(part 1 of 2)
# Autodesk Inventor assembly: robot
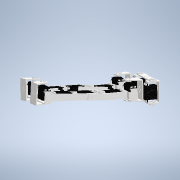
[picture p0: Inventor's stored thumbnail of the model, 180x180]
Saved by Autodesk Inventor 2021.4 (Build 254397000, 397)
## iProperties
Created: 2022-07-17
Part Number: robot
Document SubType Name: Assembly
Designer: isamu
Author: isamu
## Documents named in this file (28)
- D:\personal_projects\robot\inventor\2021-exportable\robot.iam
- D:\personal_projects\robot\exports\servo motors\servo-motor-mg996r servo.ipt
- D:\personal_projects\robot\exports\frames\servo frame.ipt
- D:\personal_projects\robot\exports\handle\servo handle 4.ipt
- D:\personal_projects\robot\exports\screws\m4x8.ipt
- D:\personal_projects\robot\exports\screws\m4 nuts.ipt
- D:\personal_projects\robot\exports\screws\m4x12.ipt
- D:\personal_projects\robot\exports\frames\servo frame mg996r.ipt
- D:\personal_projects\robot\exports\screws\m2x8.ipt
- D:\personal_projects\robot\exports\screws\m2 nuts.ipt
- D:\personal_projects\robot\exports\frames\servo frame part 3.ipt
- D:\personal_projects\robot\exports\frames\servo frame mg996 centered_MIR.ipt
- D:\personal_projects\robot\exports\frames\servo frame mg996 foot_MIR.ipt
- D:\personal_projects\robot\exports\frames\servo frame part 4.ipt
- D:\personal_projects\robot\exports\servo motors\servo-motor-mg996r servo_MIR.ipt
- D:\personal_projects\robot\exports\frames\servo frame_MIR.ipt
- D:\personal_projects\robot\exports\screws\m4x8_MIR.ipt
- D:\personal_projects\robot\exports\screws\m4 nuts_MIR.ipt
- D:\personal_projects\robot\exports\screws\m4x12_MIR.ipt
- D:\personal_projects\robot\exports\frames\servo frame mg996r_MIR.ipt
- D:\personal_projects\robot\exports\handle\servo handle 4_MIR.ipt
- D:\personal_projects\robot\exports\screws\m2x8_MIR.ipt
- D:\personal_projects\robot\exports\screws\m2 nuts_MIR.ipt
- D:\personal_projects\robot\exports\frames\servo frame part 3_MIR.ipt
- D:\personal_projects\robot\exports\frames\servo frame mg996 centered_MIR_MIR.ipt
- D:\personal_projects\robot\exports\frames\servo frame mg996 foot_MIR_MIR.ipt
- D:\personal_projects\robot\exports\screws\m3x8.ipt
- D:\personal_projects\robot\exports\screws\m3 nuts.ipt
## Components (474 placed, 27 different names)
1. servo-motor-mg996r servo:1 — Mate:1, Mate:2, Mate:3, Insert:1, Insert:2, Insert:3, Insert:4, Rotational:1
2. servo frame:1 — Mate:1, Mate:2, Mate:3, Insert:5, Insert:6, Insert:7, Insert:8, Insert:9, Insert:10, Mate:32, Mate:33, Mate:34, Insert:376, Insert:377, Insert:378, Insert:379, Insert:380
3. m4x8:1 — Insert:2
4. m4x8:2 — Insert:3
5. m4x8:3 — Insert:4
6. m4x8:4 — Insert:1
7. m4 nuts:1 — Insert:5
8. m4 nuts:2 — Insert:6
9. m4 nuts:3 — Insert:7
10. m4 nuts:4 — Insert:8
11. m4x12:1 — Insert:9
12. m4 nuts:5 — Insert:10
13. servo frame mg996r:1 — Mate:4, Mate:5, Mate:6, Insert:11, Insert:16, Insert:17, Insert:18, Insert:19, Mate:13, Mate:14, Mate:15, Mate:16, Insert:281, Insert:282, Insert:283, Insert:284, Insert:285
14. servo handle 4:1 — Rotational:1, Mate:4, Mate:5, Mate:6, Insert:12, Insert:13, Insert:14, Insert:15
15. m4 nuts:6 — Insert:11
16. m2x8:1 — Insert:12
17. m2x8:2 — Insert:13
18. m2x8:3 — Insert:15
19. m2x8:4 — Insert:14
20. m2 nuts:1 — Insert:19
21. m2 nuts:2 — Insert:18
22. m2 nuts:3 — Insert:16
23. m2 nuts:4 — Insert:17
24. servo-motor-mg996r servo:2
25. servo frame:2 — Mate:23, Mate:24, Mate:25, Insert:291, Insert:292, Insert:293, Insert:294, Insert:295
26. m4x8:5
27. m4x8:6
28. m4x8:7
29. m4x8:8
30. m4 nuts:7
31. m4 nuts:8
32. m4 nuts:9
33. m4 nuts:10
34. m4x12:2
35. m4 nuts:11
36. servo frame mg996r:2 — Mate:13, Mate:14, Mate:15, Mate:16, Insert:386, Insert:387, Insert:388, Insert:389, Insert:390
37. servo handle 4:2
38. m4 nuts:12
39. m2x8:5
40. m2x8:6
41. m2x8:7
42. m2x8:8
43. m2 nuts:5
44. m2 nuts:6
45. m2 nuts:7
46. m2 nuts:8
47. servo-motor-mg996r servo:3
48. servo frame:3 — Mate:23, Mate:24, Mate:25, Insert:396, Insert:397, Insert:398, Insert:399, Insert:400
49. m4x8:9
50. m4x8:10
51. m4x8:11
52. m4x8:12
53. m4 nuts:13
54. m4 nuts:14
55. m4 nuts:15
56. m4 nuts:16
57. m4x12:3
58. m4 nuts:17
59. servo frame mg996r:3 — Mate:44, Mate:45, Mate:46, Mate:47, Insert:296, Insert:297, Insert:298, Insert:299, Insert:300
60. servo handle 4:3
61. m4 nuts:18
62. m2x8:9
63. m2x8:10
64. m2x8:11
65. m2x8:12
66. m2 nuts:9
67. m2 nuts:10
68. m2 nuts:11
69. m2 nuts:12
70. servo-motor-mg996r servo:4
71. servo frame:4 — Mate:29, Mate:30, Mate:31, Insert:406, Insert:407, Insert:408, Insert:409, Insert:410, Insert:411, Insert:412, Insert:413, Insert:414, Insert:415
72. m4x8:13
73. m4x8:14
74. m4x8:15
75. m4x8:16
76. m4 nuts:19
77. m4 nuts:20
78. m4 nuts:21
79. m4 nuts:22
80. m4x12:4 — Mate:36
81. m4 nuts:23
82. servo handle 4:4 — Mate:35
83. m2x8:13
84. m2x8:14
85. m2x8:15
86. m2x8:16 — Mate:37
87. servo frame part 3:1 — Mate:29, Mate:30, Mate:31, Mate:32, Mate:33, Mate:34, Insert:286, Insert:287, Insert:288, Insert:289, Insert:290, Insert:316, Insert:317, Insert:318, Insert:319, Insert:320, Insert:321, Insert:322, Insert:323, Insert:324, Insert:325
88. servo frame mg996 centered_MIR:1 — Mate:35, Mate:36, Mate:37, Mate:54, Mate:55, Mate:56, Mate:146, Insert:456, Insert:468, Insert:469, Insert:470, Insert:471, Insert:476, Insert:477, Insert:478, Insert:479
89. servo-motor-mg996r servo:5
90. servo frame:5 — Mate:41, Mate:42, Mate:43, Insert:436, Insert:437, Insert:438, Insert:439, Insert:440, Insert:446, Insert:447, Insert:448, Insert:449, Insert:450
91. m4x8:17
92. m4x8:18
93. m4x8:19
94. m4x8:20
95. m4 nuts:24
96. m4 nuts:25
97. m4 nuts:26
98. m4 nuts:27
99. m4x12:5
100. m4 nuts:28
101. servo handle 4:5 — Mate:50
102. m2x8:17
103. m2x8:18 — Mate:49
104. m2x8:19 — Mate:48
105. m2x8:20
106. servo frame part 3:2 — Mate:41, Mate:42, Mate:43, Mate:44, Mate:45, Mate:46, Mate:47, Insert:346, Insert:347, Insert:348, Insert:349, Insert:350, Insert:351, Insert:352, Insert:353, Insert:354, Insert:355, Insert:426, Insert:430, Insert:431, Insert:432, Insert:433
107. servo frame mg996 foot_MIR:1 — Mate:48, Mate:49, Mate:50, Insert:458, Insert:460, Insert:461, Insert:462, Insert:463
108. servo-motor-mg996r servo:6
109. servo frame:6 — Mate:57, Mate:58, Mate:59, Mate:60, Mate:61, Mate:62, Insert:356, Insert:357, Insert:358, Insert:359, Insert:360, Insert:361, Insert:362, Insert:363, Insert:364, Insert:365
110. m4x8:21
111. m4x8:22
112. m4x8:23
113. m4x8:24
114. m4 nuts:29
115. m4 nuts:30
116. m4 nuts:31
117. m4 nuts:32
118. servo handle 4:6 — Mate:54
119. m2x8:21 — Mate:56
120. m2x8:22
121. m2x8:23 — Mate:146
122. m2x8:24 — Mate:55
123. servo frame part 4:1 — Mate:57, Mate:58, Mate:59, Mate:91, Mate:92, Mate:93, Insert:256, Insert:257, Insert:258, Insert:259, Insert:260, Insert:271, Insert:272, Insert:273, Insert:274, Insert:275
124. servo frame part 4:2 — Mate:60, Mate:61, Mate:62, Insert:261, Insert:262, Insert:263, Insert:264, Insert:265, Insert:266, Insert:267, Insert:268, Insert:269, Insert:270
125. servo-motor-mg996r servo:10
126. servo frame:10 — Mate:91, Mate:92, Mate:93, Insert:366, Insert:367, Insert:368, Insert:369, Insert:370, Insert:371, Insert:372, Insert:373, Insert:374, Insert:375
127. m4x8:37
128. m4x8:38
129. m4x8:39
130. m4x8:40
131. m4 nuts:51
132. m4 nuts:52
133. m4 nuts:53
134. m4 nuts:54
135. servo handle 4:10 — Mate:144, Insert:252, Insert:253, Insert:254, Insert:255
136. servo-motor-mg996r servo_MIR:1 — Mate:94, Mate:95, Mate:96, Insert:167, Insert:168, Insert:169, Insert:170, Rotational:11
137. servo frame_MIR:1 — Mate:94, Mate:95, Mate:96, Insert:171, Insert:172, Insert:173, Insert:174, Insert:175, Insert:176, Mate:122, Mate:123, Mate:124, Insert:381, Insert:382, Insert:383, Insert:384, Insert:385
138. m4x8_MIR:1 — Insert:167
139. m4x8_MIR:2 — Insert:168
140. m4x8_MIR:3 — Insert:169
141. m4x8_MIR:4 — Insert:170
142. m4 nuts_MIR:1 — Insert:171
143. m4 nuts_MIR:2 — Insert:172
144. m4 nuts_MIR:3 — Insert:173
145. m4 nuts_MIR:4 — Insert:174
146. m4x12_MIR:1 — Insert:175
147. m4 nuts_MIR:5 — Insert:176
148. servo frame mg996r_MIR:1 — Mate:97, Mate:98, Mate:99, Insert:177, Insert:182, Insert:183, Insert:184, Insert:185, Mate:103, Mate:104, Mate:105, Mate:106, Insert:276, Insert:277, Insert:278, Insert:279, Insert:280
149. servo handle 4_MIR:1 — Mate:97, Mate:98, Mate:99, Insert:178, Insert:179, Insert:180, Insert:181, Rotational:11
150. m4 nuts_MIR:6 — Insert:177
151. m2x8_MIR:1 — Insert:178
152. m2x8_MIR:2 — Insert:179
153. m2x8_MIR:3 — Insert:180
154. m2x8_MIR:4 — Insert:181
155. m2 nuts_MIR:1 — Insert:182
156. m2 nuts_MIR:2 — Insert:183
157. m2 nuts_MIR:3 — Insert:184
158. m2 nuts_MIR:4 — Insert:185
159. servo-motor-mg996r servo_MIR:2 — Mate:100, Mate:101, Mate:102, Insert:186, Insert:187, Insert:188, Insert:189, Rotational:12
160. servo frame_MIR:2 — Mate:100, Mate:101, Mate:102, Insert:190, Insert:191, Insert:192, Insert:193, Insert:194, Insert:195, Mate:110, Mate:111, Mate:112, Insert:306, Insert:307, Insert:308, Insert:309, Insert:310
161. m4x8_MIR:5 — Insert:186
162. m4x8_MIR:6 — Insert:187
163. m4x8_MIR:7 — Insert:188
164. m4x8_MIR:8 — Insert:189
165. m4 nuts_MIR:7 — Insert:190
166. m4 nuts_MIR:8 — Insert:191
167. m4 nuts_MIR:9 — Insert:192
168. m4 nuts_MIR:10 — Insert:193
169. m4x12_MIR:2 — Insert:194
170. m4 nuts_MIR:11 — Insert:195
171. servo frame mg996r_MIR:2 — Mate:103, Mate:104, Mate:105, Mate:106, Mate:107, Mate:108, Mate:109, Insert:196, Insert:201, Insert:202, Insert:203, Insert:204, Insert:391, Insert:392, Insert:393, Insert:394, Insert:395
172. servo handle 4_MIR:2 — Mate:107, Mate:108, Mate:109, Insert:197, Insert:198, Insert:199, Insert:200, Rotational:12
173. m4 nuts_MIR:12 — Insert:196
174. m2x8_MIR:5 — Insert:197
175. m2x8_MIR:6 — Insert:198
176. m2x8_MIR:7 — Insert:199
177. m2x8_MIR:8 — Insert:200
178. m2 nuts_MIR:5 — Insert:201
179. m2 nuts_MIR:6 — Insert:202
180. m2 nuts_MIR:7 — Insert:203
181. m2 nuts_MIR:8 — Insert:204
182. servo-motor-mg996r servo_MIR:3 — Mate:113, Mate:114, Mate:115, Insert:205, Insert:206, Insert:207, Insert:208, Rotational:13
183. servo frame_MIR:3 — Mate:110, Mate:111, Mate:112, Mate:113, Mate:114, Mate:115, Insert:209, Insert:210, Insert:211, Insert:212, Insert:213, Insert:214, Insert:401, Insert:402, Insert:403, Insert:404, Insert:405
184. m4x8_MIR:9 — Insert:205
185. m4x8_MIR:10 — Insert:206
186. m4x8_MIR:11 — Insert:207
187. m4x8_MIR:12 — Insert:208
188. m4 nuts_MIR:13 — Insert:209
189. m4 nuts_MIR:14 — Insert:210
190. m4 nuts_MIR:15 — Insert:211
191. m4 nuts_MIR:16 — Insert:212
192. m4x12_MIR:3 — Insert:213
193. m4 nuts_MIR:17 — Insert:214
194. servo frame mg996r_MIR:3 — Mate:116, Mate:117, Mate:118, Insert:215, Insert:220, Insert:221, Insert:222, Insert:223, Mate:134, Mate:135, Mate:136, Mate:137, Insert:301, Insert:302, Insert:303, Insert:304, Insert:305
195. servo handle 4_MIR:3 — Mate:116, Mate:117, Mate:118, Insert:216, Insert:217, Insert:218, Insert:219, Rotational:13
196. m4 nuts_MIR:18 — Insert:215
197. m2x8_MIR:9 — Insert:216
198. m2x8_MIR:10 — Insert:217
199. m2x8_MIR:11 — Insert:218
200. m2x8_MIR:12 — Insert:219
201. m2 nuts_MIR:9 — Insert:220
202. m2 nuts_MIR:10 — Insert:221
203. m2 nuts_MIR:11 — Insert:222
204. m2 nuts_MIR:12 — Insert:223
205. servo-motor-mg996r servo_MIR:4 — Mate:119, Mate:120, Mate:121, Insert:224, Insert:225, Insert:226, Insert:227, Rotational:14
206. servo frame_MIR:4 — Mate:119, Mate:120, Mate:121, Insert:228, Insert:229, Insert:230, Insert:231, Insert:232, Insert:233, Mate:125, Mate:126, Mate:127, Insert:416, Insert:417, Insert:418, Insert:419, Insert:420, Insert:421, Insert:422, Insert:423, Insert:424, Insert:425
207. m4x8_MIR:13 — Insert:224
208. m4x8_MIR:14 — Insert:225
209. m4x8_MIR:15 — Insert:226
210. m4x8_MIR:16 — Insert:227
211. m4 nuts_MIR:19 — Insert:228
212. m4 nuts_MIR:20 — Insert:229
213. m4 nuts_MIR:21 — Insert:230
214. m4 nuts_MIR:22 — Insert:231
215. m4x12_MIR:4 — Insert:232, Mate:129
216. m4 nuts_MIR:23 — Insert:233
217. servo handle 4_MIR:4 — Insert:234, Insert:235, Insert:236, Insert:237, Mate:130, Rotational:14
218. m2x8_MIR:13 — Insert:234
219. m2x8_MIR:14 — Insert:235
220. m2x8_MIR:15 — Insert:236
221. m2x8_MIR:16 — Insert:237, Mate:128
222. servo frame part 3_MIR:1 — Mate:122, Mate:123, Mate:124, Mate:125, Mate:126, Mate:127, Insert:311, Insert:312, Insert:313, Insert:314, Insert:315, Insert:326, Insert:327, Insert:328, Insert:329, Insert:330, Insert:331, Insert:332, Insert:333, Insert:334, Insert:335
223. servo frame mg996 centered_MIR_MIR:1 — Mate:128, Mate:129, Mate:130, Mate:144, Mate:147, Mate:148, Insert:457, Insert:472, Insert:473, Insert:474, Insert:475, Insert:480, Insert:481, Insert:482, Insert:483
224. servo-motor-mg996r servo_MIR:5 — Mate:131, Mate:132, Mate:133, Insert:238, Insert:239, Insert:240, Insert:241, Rotational:15
225. servo frame_MIR:5 — Mate:131, Mate:132, Mate:133, Insert:242, Insert:243, Insert:244, Insert:245, Insert:246, Insert:247, Mate:138, Mate:139, Mate:140, Insert:441, Insert:442, Insert:443, Insert:444, Insert:445, Insert:451, Insert:452, Insert:453, Insert:454, Insert:455
226. m4x8_MIR:17 — Insert:238
227. m4x8_MIR:18 — Insert:239
228. m4x8_MIR:19 — Insert:240
229. m4x8_MIR:20 — Insert:241
230. m4 nuts_MIR:24 — Insert:242
231. m4 nuts_MIR:25 — Insert:243
232. m4 nuts_MIR:26 — Insert:244
233. m4 nuts_MIR:27 — Insert:245
234. m4x12_MIR:5 — Insert:246
235. m4 nuts_MIR:28 — Insert:247
236. servo handle 4_MIR:5 — Insert:248, Insert:249, Insert:250, Insert:251, Mate:141, Rotational:15
237. m2x8_MIR:17 — Insert:248
238. m2x8_MIR:18 — Insert:249, Mate:142
239. m2x8_MIR:19 — Insert:250, Mate:143
240. m2x8_MIR:20 — Insert:251
241. servo frame part 3_MIR:2 — Mate:134, Mate:135, Mate:136, Mate:137, Mate:138, Mate:139, Mate:140, Insert:336, Insert:337, Insert:338, Insert:339, Insert:340, Insert:341, Insert:342, Insert:343, Insert:344, Insert:345, Insert:427, Insert:428, Insert:429, Insert:434, Insert:435
242. servo frame mg996 foot_MIR_MIR:1 — Mate:141, Mate:142, Mate:143, Insert:459, Insert:464, Insert:465, Insert:466, Insert:467
243. m2x8:41 — Insert:252
244. m2x8:42 — Insert:255, Mate:148
245. m2x8:43 — Insert:253, Mate:147
246. m2x8:44 — Insert:254
247. m3x8:1 — Insert:269
248. m3x8:2 — Insert:270
249. m3x8:3 — Insert:265
250. m3x8:4 — Insert:264
251. m3x8:5 — Insert:266
252. m3x8:6 — Insert:276
253. m3x8:7 — Insert:277
254. m3x8:8 — Insert:278
255. m3x8:9 — Insert:274
256. m3x8:10 — Insert:275
257. m3x8:11 — Insert:271
258. m3x8:12 — Insert:284
259. m3x8:13 — Insert:283
260. m3x8:14 — Insert:282
261. m3x8:15 — Insert:281
262. m3x8:16 — Insert:259
263. m3x8:17 — Insert:260
264. m3x8:18 — Insert:258
265. m3x8:19 — Insert:257
266. m3x8:20 — Insert:256
267. m3x8:21 — Insert:280
268. m3x8:22 — Insert:285
269. m3x8:23 — Insert:279
270. m3x8:24 — Insert:272
271. m3x8:25 — Insert:273
272. m3x8:26 — Insert:290
273. m3x8:27 — Insert:289
274. m3x8:28 — Insert:288
275. m3x8:29 — Insert:287
276. m3x8:30 — Insert:286
277. m3x8:31 — Insert:306
278. m3x8:32 — Insert:330
279. m3x8:33 — Insert:329
280. m3x8:34 — Insert:311
281. m3x8:35 — Insert:342
282. m3x8:36 — Insert:263
283. m3x8:37 — Insert:268
284. m3x8:38 — Insert:267
285. m3x8:39 — Insert:262
286. m3x8:40 — Insert:261
287. m3x8:41 — Insert:298
288. m3x8:42 — Insert:300
289. m3x8:43 — Insert:299
290. m3x8:44 — Insert:301
291. m3x8:45 — Insert:305
292. m3x8:46 — Insert:307
293. m3x8:47 — Insert:312
294. m3x8:48 — Insert:313
295. m3x8:49 — Insert:315
296. m3x8:50 — Insert:314
297. m3x8:51 — Insert:296
298. m3x8:52 — Insert:297
299. m3x8:53 — Insert:308
300. m3x8:54 — Insert:309
301. m3x8:55 — Insert:310
302. m3x8:56 — Insert:340
303. m3x8:57 — Insert:341
304. m3x8:58 — Insert:328
305. m3x8:59 — Insert:327
306. m3x8:60 — Insert:326
307. m3x8:61 — Insert:303
308. m3x8:62 — Insert:336
309. m3x8:63 — Insert:337
310. m3x8:64 — Insert:304
311. m3x8:65 — Insert:302
312. m3x8:66 — Insert:291
313. m3x8:67 — Insert:292
314. m3x8:68 — Insert:293
315. m3x8:69 — Insert:294
316. m3x8:70 — Insert:295
317. m3x8:71 — Insert:321
318. m3x8:72 — Insert:323
319. m3x8:73 — Insert:325
320. m3x8:74 — Insert:318
321. m3x8:75 — Insert:322
322. m3x8:76 — Insert:324
323. m3x8:77 — Insert:320
324. m3x8:78 — Insert:319
325. m3x8:79 — Insert:317
326. m3x8:80 — Insert:316
327. m3x8:81 — Insert:344
328. m3x8:82 — Insert:343
329. m3x8:83 — Insert:345
330. m3x8:84 — Insert:338
331. m3x8:85 — Insert:339
332. m3x8:86 — Insert:353
333. m3x8:87 — Insert:350
334. m3x8:88 — Insert:354
335. m3x8:89 — Insert:347
336. m3x8:90 — Insert:348
337. m3x8:91 — Insert:352
338. m3x8:92 — Insert:355
339. m3x8:93 — Insert:351
340. m3x8:94 — Insert:349
341. m3x8:95 — Insert:346
342. m3x8:96 — Insert:335
343. m3x8:97 — Insert:334
344. m3x8:98 — Insert:331
345. m3x8:99 — Insert:332
346. m3x8:100 — Insert:333
347. m3 nuts:1 — Insert:358
348. m3 nuts:2 — Insert:359
349. m3 nuts:3 — Insert:365
350. m3 nuts:4 — Insert:361
351. m3 nuts:5 — Insert:362
352. m3 nuts:6 — Insert:356
353. m3 nuts:7 — Insert:357
354. m3 nuts:8 — Insert:360
355. m3 nuts:9 — Insert:363
356. m3 nuts:10 — Insert:364
357. m3 nuts:11 — Insert:389
358. m3 nuts:12 — Insert:394
359. m3 nuts:13 — Insert:385
360. m3 nuts:14 — Insert:401
361. m3 nuts:15 — Insert:440
362. m3 nuts:16 — Insert:392
363. m3 nuts:17 — Insert:369
364. m3 nuts:18 — Insert:379
365. m3 nuts:19 — Insert:390
366. m3 nuts:20 — Insert:433
367. m3 nuts:21 — Insert:398
368. m3 nuts:22 — Insert:381
369. m3 nuts:23 — Insert:367
370. m3 nuts:24 — Insert:371
371. m3 nuts:25 — Insert:391
372. m3 nuts:26 — Insert:397
373. m3 nuts:27 — Insert:402
374. m3 nuts:28 — Insert:386
375. m3 nuts:29 — Insert:376
376. m3 nuts:30 — Insert:380
377. m3 nuts:31 — Insert:399
378. m3 nuts:32 — Insert:404
379. m3 nuts:33 — Insert:372
380. m3 nuts:34 — Insert:370
381. m3 nuts:35 — Insert:366
382. m3 nuts:36 — Insert:400
383. m3 nuts:37 — Insert:403
384. m3 nuts:38 — Insert:387
385. m3 nuts:39 — Insert:368
386. m3 nuts:40 — Insert:373
387. m3 nuts:41 — Insert:375
388. m3 nuts:42 — Insert:395
389. m3 nuts:43 — Insert:396
390. m3 nuts:44 — Insert:393
391. m3 nuts:45 — Insert:388
392. m3 nuts:46 — Insert:378
393. m3 nuts:47 — Insert:384
394. m3 nuts:48 — Insert:423
395. m3 nuts:49 — Insert:415
396. m3 nuts:50 — Insert:438
397. m3 nuts:51 — Insert:377
398. m3 nuts:52 — Insert:383
399. m3 nuts:53 — Insert:382
400. m3 nuts:54 — Insert:439
401. m3 nuts:55 — Insert:454
402. m3 nuts:56 — Insert:426
403. m3 nuts:57 — Insert:432
404. m3 nuts:58 — Insert:452
405. m3 nuts:59 — Insert:455
406. m3 nuts:60 — Insert:431
407. m3 nuts:61 — Insert:425
408. m3 nuts:62 — Insert:420
409. m3 nuts:63 — Insert:422
410. m3 nuts:64 — Insert:451
411. m3 nuts:65 — Insert:453
412. m3 nuts:66 — Insert:430
413. m3 nuts:67 — Insert:416
414. m3 nuts:68 — Insert:414
415. m3 nuts:69 — Insert:435
416. m3 nuts:70 — Insert:437
417. m3 nuts:71 — Insert:436
418. m3 nuts:72 — Insert:427
419. m3 nuts:73 — Insert:406
420. m3 nuts:74 — Insert:411
421. m3 nuts:75 — Insert:421
422. m3 nuts:76 — Insert:429
423. m3 nuts:77 — Insert:419
424. m3 nuts:78 — Insert:410
425. m3 nuts:79 — Insert:405
426. m3 nuts:80 — Insert:409
427. m3 nuts:81 — Insert:417
428. m3 nuts:82 — Insert:418
429. m3 nuts:83 — Insert:407
430. m3 nuts:84 — Insert:408
431. m3 nuts:85 — Insert:412
432. m3 nuts:86 — Insert:413
433. m3 nuts:87 — Insert:424
434. m3 nuts:88 — Insert:434
435. m3 nuts:89 — Insert:428
436. m3 nuts:90 — Insert:374
437. m3 nuts:91 — Insert:445
438. m3 nuts:92 — Insert:444
439. m3 nuts:93 — Insert:442
440. m3 nuts:94 — Insert:443
441. m3 nuts:95 — Insert:441
442. m3 nuts:96 — Insert:447
443. m3 nuts:97 — Insert:449
444. m3 nuts:98 — Insert:448
445. m3 nuts:99 — Insert:446
446. m3 nuts:100 — Insert:450
447. m4 nuts:55 — Insert:458
448. m4 nuts:56 — Insert:456
449. m4 nuts:57 — Insert:457
450. m4 nuts:58 — Insert:459
451. m2 nuts:13 — Insert:464
452. m2 nuts:14 — Insert:465
453. m2 nuts:15 — Insert:463
454. m2 nuts:16 — Insert:462
455. m2 nuts:17 — Insert:477
456. m2 nuts:18 — Insert:470
457. m2 nuts:19 — Insert:461
458. m2 nuts:20 — Insert:460
459. m2 nuts:21 — Insert:468
460. m2 nuts:22 — Insert:480
461. m2 nuts:23 — Insert:483
462. m2 nuts:24 — Insert:481
463. m2 nuts:25 — Insert:471
464. m2 nuts:26 — Insert:475
465. m2 nuts:27 — Insert:472
466. m2 nuts:28 — Insert:482
467. m2 nuts:29 — Insert:479
468. m2 nuts:30 — Insert:478
469. m2 nuts:31 — Insert:476
470. m2 nuts:32 — Insert:469
471. m2 nuts:33 — Insert:466
472. m2 nuts:34 — Insert:473
473. m2 nuts:35 — Insert:474
474. m2 nuts:36 — Insert:467
## Relationships (556: Insert 422, Mate 122, RevoluteJoint 12)
- Mate:1: servo-motor-mg996r servo:1 ↔ servo frame:1
- Mate:2: servo-motor-mg996r servo:1 ↔ servo frame:1
- Mate:3: servo-motor-mg996r servo:1 ↔ servo frame:1
- Insert:1: servo-motor-mg996r servo:1 ↔ m4x8:4
- Insert:2: servo-motor-mg996r servo:1 ↔ m4x8:1
- Insert:3: servo-motor-mg996r servo:1 ↔ m4x8:2
- Insert:4: servo-motor-mg996r servo:1 ↔ m4x8:3
- Insert:5: servo frame:1 ↔ m4 nuts:1
- Insert:6: servo frame:1 ↔ m4 nuts:2
- Insert:7: servo frame:1 ↔ m4 nuts:3
- Insert:8: servo frame:1 ↔ m4 nuts:4
- Insert:9: servo frame:1 ↔ m4x12:1
- Insert:10: servo frame:1 ↔ m4 nuts:5
- Mate:4: servo frame mg996r:1 ↔ servo handle 4:1
- Mate:5: servo frame mg996r:1 ↔ servo handle 4:1
- Mate:6: servo frame mg996r:1 ↔ servo handle 4:1
- Insert:11: servo frame mg996r:1 ↔ m4 nuts:6
- Insert:12: servo handle 4:1 ↔ m2x8:1
- Insert:13: servo handle 4:1 ↔ m2x8:2
- Insert:14: servo handle 4:1 ↔ m2x8:4
- Insert:15: servo handle 4:1 ↔ m2x8:3
- Insert:16: servo frame mg996r:1 ↔ m2 nuts:3
- Insert:17: servo frame mg996r:1 ↔ m2 nuts:4
- Insert:18: servo frame mg996r:1 ↔ m2 nuts:2
- Insert:19: servo frame mg996r:1 ↔ m2 nuts:1
- [Mate]: servo-motor-mg996r servo:2 ↔ servo frame:2
- [Mate]: servo-motor-mg996r servo:2 ↔ servo frame:2
- [Mate]: servo-motor-mg996r servo:2 ↔ servo frame:2
- [Insert]: servo-motor-mg996r servo:2 ↔ m4x8:8
- [Insert]: servo-motor-mg996r servo:2 ↔ m4x8:5
- [Insert]: servo-motor-mg996r servo:2 ↔ m4x8:6
- [Insert]: servo-motor-mg996r servo:2 ↔ m4x8:7
- [Insert]: servo frame:2 ↔ m4 nuts:7
- [Insert]: servo frame:2 ↔ m4 nuts:8
- [Insert]: servo frame:2 ↔ m4 nuts:9
- [Insert]: servo frame:2 ↔ m4 nuts:10
- [Insert]: servo frame:2 ↔ m4x12:2
- [Insert]: servo frame:2 ↔ m4 nuts:11
- [Mate]: servo frame mg996r:2 ↔ servo handle 4:2
- [Mate]: servo frame mg996r:2 ↔ servo handle 4:2
- [Mate]: servo frame mg996r:2 ↔ servo handle 4:2
- [Insert]: servo frame mg996r:2 ↔ m4 nuts:12
- [Insert]: servo handle 4:2 ↔ m2x8:5
- [Insert]: servo handle 4:2 ↔ m2x8:6
- [Insert]: servo handle 4:2 ↔ m2x8:8
- [Insert]: servo handle 4:2 ↔ m2x8:7
- [Insert]: servo frame mg996r:2 ↔ m2 nuts:7
- [Insert]: servo frame mg996r:2 ↔ m2 nuts:8
- [Insert]: servo frame mg996r:2 ↔ m2 nuts:6
- [Insert]: servo frame mg996r:2 ↔ m2 nuts:5
- Mate:13: servo frame mg996r:1 ↔ servo frame mg996r:2
- Mate:14: servo frame mg996r:1 ↔ servo frame mg996r:2
- Mate:15: servo frame mg996r:1 ↔ servo frame mg996r:2
- Mate:16: servo frame mg996r:1 ↔ servo frame mg996r:2
- [Mate]: servo-motor-mg996r servo:3 ↔ servo frame:3
- [Mate]: servo-motor-mg996r servo:3 ↔ servo frame:3
- [Mate]: servo-motor-mg996r servo:3 ↔ servo frame:3
- [Insert]: servo-motor-mg996r servo:3 ↔ m4x8:12
- [Insert]: servo-motor-mg996r servo:3 ↔ m4x8:9
- [Insert]: servo-motor-mg996r servo:3 ↔ m4x8:10
- [Insert]: servo-motor-mg996r servo:3 ↔ m4x8:11
- [Insert]: servo frame:3 ↔ m4 nuts:13
- [Insert]: servo frame:3 ↔ m4 nuts:14
- [Insert]: servo frame:3 ↔ m4 nuts:15
- [Insert]: servo frame:3 ↔ m4 nuts:16
- [Insert]: servo frame:3 ↔ m4x12:3
- [Insert]: servo frame:3 ↔ m4 nuts:17
- [Mate]: servo frame mg996r:3 ↔ servo handle 4:3
- [Mate]: servo frame mg996r:3 ↔ servo handle 4:3
- [Mate]: servo frame mg996r:3 ↔ servo handle 4:3
- [Insert]: servo frame mg996r:3 ↔ m4 nuts:18
- [Insert]: servo handle 4:3 ↔ m2x8:9
- [Insert]: servo handle 4:3 ↔ m2x8:10
- [Insert]: servo handle 4:3 ↔ m2x8:12
- [Insert]: servo handle 4:3 ↔ m2x8:11
- [Insert]: servo frame mg996r:3 ↔ m2 nuts:11
- [Insert]: servo frame mg996r:3 ↔ m2 nuts:12
- [Insert]: servo frame mg996r:3 ↔ m2 nuts:10
- [Insert]: servo frame mg996r:3 ↔ m2 nuts:9
- Mate:23: servo frame:2 ↔ servo frame:3
- Mate:24: servo frame:2 ↔ servo frame:3
- Mate:25: servo frame:2 ↔ servo frame:3
- [Mate]: servo-motor-mg996r servo:4 ↔ servo frame:4
- [Mate]: servo-motor-mg996r servo:4 ↔ servo frame:4
- [Mate]: servo-motor-mg996r servo:4 ↔ servo frame:4
- [Insert]: servo-motor-mg996r servo:4 ↔ m4x8:16
- [Insert]: servo-motor-mg996r servo:4 ↔ m4x8:13
- [Insert]: servo-motor-mg996r servo:4 ↔ m4x8:14
- [Insert]: servo-motor-mg996r servo:4 ↔ m4x8:15
- [Insert]: servo frame:4 ↔ m4 nuts:19
- [Insert]: servo frame:4 ↔ m4 nuts:20
- [Insert]: servo frame:4 ↔ m4 nuts:21
- [Insert]: servo frame:4 ↔ m4 nuts:22
- [Insert]: servo frame:4 ↔ m4x12:4
- [Insert]: servo frame:4 ↔ m4 nuts:23
- [Insert]: servo handle 4:4 ↔ m2x8:13
- [Insert]: servo handle 4:4 ↔ m2x8:14
- [Insert]: servo handle 4:4 ↔ m2x8:16
- [Insert]: servo handle 4:4 ↔ m2x8:15
- Mate:29: servo frame:4 ↔ servo frame part 3:1
- Mate:30: servo frame:4 ↔ servo frame part 3:1
- Mate:31: servo frame:4 ↔ servo frame part 3:1
- Mate:32: servo frame:1 ↔ servo frame part 3:1
- Mate:33: servo frame:1 ↔ servo frame part 3:1
- Mate:34: servo frame:1 ↔ servo frame part 3:1
- Mate:35: servo handle 4:4 ↔ servo frame mg996 centered_MIR:1
- Mate:36: m4x12:4 ↔ servo frame mg996 centered_MIR:1
- Mate:37: m2x8:16 ↔ servo frame mg996 centered_MIR:1
- [Mate]: servo-motor-mg996r servo:5 ↔ servo frame:5
- [Mate]: servo-motor-mg996r servo:5 ↔ servo frame:5
- [Mate]: servo-motor-mg996r servo:5 ↔ servo frame:5
- [Insert]: servo-motor-mg996r servo:5 ↔ m4x8:20
- [Insert]: servo-motor-mg996r servo:5 ↔ m4x8:17
- [Insert]: servo-motor-mg996r servo:5 ↔ m4x8:18
- [Insert]: servo-motor-mg996r servo:5 ↔ m4x8:19
- [Insert]: servo frame:5 ↔ m4 nuts:24
- [Insert]: servo frame:5 ↔ m4 nuts:25
- [Insert]: servo frame:5 ↔ m4 nuts:26
- [Insert]: servo frame:5 ↔ m4 nuts:27
- [Insert]: servo frame:5 ↔ m4x12:5
- [Insert]: servo frame:5 ↔ m4 nuts:28
- [Insert]: servo handle 4:5 ↔ m2x8:17
- [Insert]: servo handle 4:5 ↔ m2x8:18
- [Insert]: servo handle 4:5 ↔ m2x8:20
- [Insert]: servo handle 4:5 ↔ m2x8:19
- Mate:41: servo frame:5 ↔ servo frame part 3:2
- Mate:42: servo frame:5 ↔ servo frame part 3:2
- Mate:43: servo frame:5 ↔ servo frame part 3:2
- Mate:44: servo frame mg996r:3 ↔ servo frame part 3:2
- Mate:45: servo frame mg996r:3 ↔ servo frame part 3:2
- Mate:46: servo frame mg996r:3 ↔ servo frame part 3:2
- Mate:47: servo frame mg996r:3 ↔ servo frame part 3:2
- Mate:48: m2x8:19 ↔ servo frame mg996 foot_MIR:1
- Mate:49: m2x8:18 ↔ servo frame mg996 foot_MIR:1
- Mate:50: servo handle 4:5 ↔ servo frame mg996 foot_MIR:1
- [Mate]: servo-motor-mg996r servo:6 ↔ servo frame:6
- [Mate]: servo-motor-mg996r servo:6 ↔ servo frame:6
- [Mate]: servo-motor-mg996r servo:6 ↔ servo frame:6
- [Insert]: servo-motor-mg996r servo:6 ↔ m4x8:24
- [Insert]: servo-motor-mg996r servo:6 ↔ m4x8:21
- [Insert]: servo-motor-mg996r servo:6 ↔ m4x8:22
- [Insert]: servo-motor-mg996r servo:6 ↔ m4x8:23
- [Insert]: servo frame:6 ↔ m4 nuts:29
- [Insert]: servo frame:6 ↔ m4 nuts:30
- [Insert]: servo frame:6 ↔ m4 nuts:31
- [Insert]: servo frame:6 ↔ m4 nuts:32
- [Insert]: servo handle 4:6 ↔ m2x8:21
- [Insert]: servo handle 4:6 ↔ m2x8:22
- [Insert]: servo handle 4:6 ↔ m2x8:24
- [Insert]: servo handle 4:6 ↔ m2x8:23
- Mate:54: servo frame mg996 centered_MIR:1 ↔ servo handle 4:6
- Mate:55: servo frame mg996 centered_MIR:1 ↔ m2x8:24
- Mate:56: servo frame mg996 centered_MIR:1 ↔ m2x8:21
- Mate:57: servo frame:6 ↔ servo frame part 4:1
- Mate:58: servo frame:6 ↔ servo frame part 4:1
- Mate:59: servo frame:6 ↔ servo frame part 4:1
- Mate:60: servo frame:6 ↔ servo frame part 4:2
- Mate:61: servo frame:6 ↔ servo frame part 4:2
- Mate:62: servo frame:6 ↔ servo frame part 4:2
- [Mate]: servo-motor-mg996r servo:10 ↔ servo frame:10
- [Mate]: servo-motor-mg996r servo:10 ↔ servo frame:10
- [Mate]: servo-motor-mg996r servo:10 ↔ servo frame:10
- [Insert]: servo-motor-mg996r servo:10 ↔ m4x8:40
- [Insert]: servo-motor-mg996r servo:10 ↔ m4x8:37
- [Insert]: servo-motor-mg996r servo:10 ↔ m4x8:38
- [Insert]: servo-motor-mg996r servo:10 ↔ m4x8:39
- [Insert]: servo frame:10 ↔ m4 nuts:51
- [Insert]: servo frame:10 ↔ m4 nuts:52
- [Insert]: servo frame:10 ↔ m4 nuts:53
- [Insert]: servo frame:10 ↔ m4 nuts:54
- Mate:91: servo frame part 4:1 ↔ servo frame:10
- Mate:92: servo frame part 4:1 ↔ servo frame:10
- Mate:93: servo frame part 4:1 ↔ servo frame:10
- Mate:94: servo-motor-mg996r servo_MIR:1 ↔ servo frame_MIR:1
- Mate:95: servo-motor-mg996r servo_MIR:1 ↔ servo frame_MIR:1
- Mate:96: servo-motor-mg996r servo_MIR:1 ↔ servo frame_MIR:1
- Insert:167: servo-motor-mg996r servo_MIR:1 ↔ m4x8_MIR:1
- Insert:168: servo-motor-mg996r servo_MIR:1 ↔ m4x8_MIR:2
- Insert:169: servo-motor-mg996r servo_MIR:1 ↔ m4x8_MIR:3
- Insert:170: servo-motor-mg996r servo_MIR:1 ↔ m4x8_MIR:4
- Insert:171: servo frame_MIR:1 ↔ m4 nuts_MIR:1
- Insert:172: servo frame_MIR:1 ↔ m4 nuts_MIR:2
- Insert:173: servo frame_MIR:1 ↔ m4 nuts_MIR:3
- Insert:174: servo frame_MIR:1 ↔ m4 nuts_MIR:4
- Insert:175: servo frame_MIR:1 ↔ m4x12_MIR:1
- Insert:176: servo frame_MIR:1 ↔ m4 nuts_MIR:5
- Mate:97: servo frame mg996r_MIR:1 ↔ servo handle 4_MIR:1
- Mate:98: servo frame mg996r_MIR:1 ↔ servo handle 4_MIR:1
- Mate:99: servo frame mg996r_MIR:1 ↔ servo handle 4_MIR:1
- Insert:177: servo frame mg996r_MIR:1 ↔ m4 nuts_MIR:6
- Insert:178: servo handle 4_MIR:1 ↔ m2x8_MIR:1
- Insert:179: servo handle 4_MIR:1 ↔ m2x8_MIR:2
- Insert:180: servo handle 4_MIR:1 ↔ m2x8_MIR:3
- Insert:181: servo handle 4_MIR:1 ↔ m2x8_MIR:4
- Insert:182: servo frame mg996r_MIR:1 ↔ m2 nuts_MIR:1
- Insert:183: servo frame mg996r_MIR:1 ↔ m2 nuts_MIR:2
- Insert:184: servo frame mg996r_MIR:1 ↔ m2 nuts_MIR:3
- Insert:185: servo frame mg996r_MIR:1 ↔ m2 nuts_MIR:4
- Mate:100: servo-motor-mg996r servo_MIR:2 ↔ servo frame_MIR:2
- Mate:101: servo-motor-mg996r servo_MIR:2 ↔ servo frame_MIR:2
- Mate:102: servo-motor-mg996r servo_MIR:2 ↔ servo frame_MIR:2
- Insert:186: servo-motor-mg996r servo_MIR:2 ↔ m4x8_MIR:5
- Insert:187: servo-motor-mg996r servo_MIR:2 ↔ m4x8_MIR:6
- Insert:188: servo-motor-mg996r servo_MIR:2 ↔ m4x8_MIR:7
- Insert:189: servo-motor-mg996r servo_MIR:2 ↔ m4x8_MIR:8
- Insert:190: servo frame_MIR:2 ↔ m4 nuts_MIR:7
- Insert:191: servo frame_MIR:2 ↔ m4 nuts_MIR:8
- Insert:192: servo frame_MIR:2 ↔ m4 nuts_MIR:9
- Insert:193: servo frame_MIR:2 ↔ m4 nuts_MIR:10
- Insert:194: servo frame_MIR:2 ↔ m4x12_MIR:2
- Insert:195: servo frame_MIR:2 ↔ m4 nuts_MIR:11
- Mate:103: servo frame mg996r_MIR:1 ↔ servo frame mg996r_MIR:2
- Mate:104: servo frame mg996r_MIR:1 ↔ servo frame mg996r_MIR:2
- Mate:105: servo frame mg996r_MIR:1 ↔ servo frame mg996r_MIR:2
- Mate:106: servo frame mg996r_MIR:1 ↔ servo frame mg996r_MIR:2
- Mate:107: servo frame mg996r_MIR:2 ↔ servo handle 4_MIR:2
- Mate:108: servo frame mg996r_MIR:2 ↔ servo handle 4_MIR:2
- Mate:109: servo frame mg996r_MIR:2 ↔ servo handle 4_MIR:2
- Insert:196: servo frame mg996r_MIR:2 ↔ m4 nuts_MIR:12
- Insert:197: servo handle 4_MIR:2 ↔ m2x8_MIR:5
- Insert:198: servo handle 4_MIR:2 ↔ m2x8_MIR:6
- Insert:199: servo handle 4_MIR:2 ↔ m2x8_MIR:7
- Insert:200: servo handle 4_MIR:2 ↔ m2x8_MIR:8
- Insert:201: servo frame mg996r_MIR:2 ↔ m2 nuts_MIR:5
- Insert:202: servo frame mg996r_MIR:2 ↔ m2 nuts_MIR:6
- Insert:203: servo frame mg996r_MIR:2 ↔ m2 nuts_MIR:7
- Insert:204: servo frame mg996r_MIR:2 ↔ m2 nuts_MIR:8
- Mate:110: servo frame_MIR:2 ↔ servo frame_MIR:3
- Mate:111: servo frame_MIR:2 ↔ servo frame_MIR:3
- Mate:112: servo frame_MIR:2 ↔ servo frame_MIR:3
- Mate:113: servo-motor-mg996r servo_MIR:3 ↔ servo frame_MIR:3
- Mate:114: servo-motor-mg996r servo_MIR:3 ↔ servo frame_MIR:3
- Mate:115: servo-motor-mg996r servo_MIR:3 ↔ servo frame_MIR:3
- Insert:205: servo-motor-mg996r servo_MIR:3 ↔ m4x8_MIR:9
- Insert:206: servo-motor-mg996r servo_MIR:3 ↔ m4x8_MIR:10
- Insert:207: servo-motor-mg996r servo_MIR:3 ↔ m4x8_MIR:11
- Insert:208: servo-motor-mg996r servo_MIR:3 ↔ m4x8_MIR:12
- Insert:209: servo frame_MIR:3 ↔ m4 nuts_MIR:13
- Insert:210: servo frame_MIR:3 ↔ m4 nuts_MIR:14
- Insert:211: servo frame_MIR:3 ↔ m4 nuts_MIR:15
- Insert:212: servo frame_MIR:3 ↔ m4 nuts_MIR:16
- Insert:213: servo frame_MIR:3 ↔ m4x12_MIR:3
- Insert:214: servo frame_MIR:3 ↔ m4 nuts_MIR:17
- Mate:116: servo frame mg996r_MIR:3 ↔ servo handle 4_MIR:3
- Mate:117: servo frame mg996r_MIR:3 ↔ servo handle 4_MIR:3
- Mate:118: servo frame mg996r_MIR:3 ↔ servo handle 4_MIR:3
- Insert:215: servo frame mg996r_MIR:3 ↔ m4 nuts_MIR:18
- Insert:216: servo handle 4_MIR:3 ↔ m2x8_MIR:9
- Insert:217: servo handle 4_MIR:3 ↔ m2x8_MIR:10
- Insert:218: servo handle 4_MIR:3 ↔ m2x8_MIR:11
- Insert:219: servo handle 4_MIR:3 ↔ m2x8_MIR:12
- Insert:220: servo frame mg996r_MIR:3 ↔ m2 nuts_MIR:9
- Insert:221: servo frame mg996r_MIR:3 ↔ m2 nuts_MIR:10
- Insert:222: servo frame mg996r_MIR:3 ↔ m2 nuts_MIR:11
- Insert:223: servo frame mg996r_MIR:3 ↔ m2 nuts_MIR:12
- Mate:119: servo-motor-mg996r servo_MIR:4 ↔ servo frame_MIR:4
- Mate:120: servo-motor-mg996r servo_MIR:4 ↔ servo frame_MIR:4
- Mate:121: servo-motor-mg996r servo_MIR:4 ↔ servo frame_MIR:4
- Insert:224: servo-motor-mg996r servo_MIR:4 ↔ m4x8_MIR:13
- Insert:225: servo-motor-mg996r servo_MIR:4 ↔ m4x8_MIR:14
- Insert:226: servo-motor-mg996r servo_MIR:4 ↔ m4x8_MIR:15
- Insert:227: servo-motor-mg996r servo_MIR:4 ↔ m4x8_MIR:16
- Insert:228: servo frame_MIR:4 ↔ m4 nuts_MIR:19
- Insert:229: servo frame_MIR:4 ↔ m4 nuts_MIR:20
- Insert:230: servo frame_MIR:4 ↔ m4 nuts_MIR:21
- Insert:231: servo frame_MIR:4 ↔ m4 nuts_MIR:22
- Insert:232: servo frame_MIR:4 ↔ m4x12_MIR:4
- Insert:233: servo frame_MIR:4 ↔ m4 nuts_MIR:23
- Insert:234: servo handle 4_MIR:4 ↔ m2x8_MIR:13
- Insert:235: servo handle 4_MIR:4 ↔ m2x8_MIR:14
- Insert:236: servo handle 4_MIR:4 ↔ m2x8_MIR:15
- Insert:237: servo handle 4_MIR:4 ↔ m2x8_MIR:16
- Mate:122: servo frame_MIR:1 ↔ servo frame part 3_MIR:1
- Mate:123: servo frame_MIR:1 ↔ servo frame part 3_MIR:1
- Mate:124: servo frame_MIR:1 ↔ servo frame part 3_MIR:1
- Mate:125: servo frame_MIR:4 ↔ servo frame part 3_MIR:1
- Mate:126: servo frame_MIR:4 ↔ servo frame part 3_MIR:1
- Mate:127: servo frame_MIR:4 ↔ servo frame part 3_MIR:1
- Mate:128: m2x8_MIR:16 ↔ servo frame mg996 centered_MIR_MIR:1
- Mate:129: m4x12_MIR:4 ↔ servo frame mg996 centered_MIR_MIR:1
- Mate:130: servo handle 4_MIR:4 ↔ servo frame mg996 centered_MIR_MIR:1
- Mate:131: servo-motor-mg996r servo_MIR:5 ↔ servo frame_MIR:5
- Mate:132: servo-motor-mg996r servo_MIR:5 ↔ servo frame_MIR:5
- Mate:133: servo-motor-mg996r servo_MIR:5 ↔ servo frame_MIR:5
- Insert:238: servo-motor-mg996r servo_MIR:5 ↔ m4x8_MIR:17
- Insert:239: servo-motor-mg996r servo_MIR:5 ↔ m4x8_MIR:18
- Insert:240: servo-motor-mg996r servo_MIR:5 ↔ m4x8_MIR:19
- Insert:241: servo-motor-mg996r servo_MIR:5 ↔ m4x8_MIR:20
- Insert:242: servo frame_MIR:5 ↔ m4 nuts_MIR:24
- Insert:243: servo frame_MIR:5 ↔ m4 nuts_MIR:25
- Insert:244: servo frame_MIR:5 ↔ m4 nuts_MIR:26
- Insert:245: servo frame_MIR:5 ↔ m4 nuts_MIR:27
- Insert:246: servo frame_MIR:5 ↔ m4x12_MIR:5
- Insert:247: servo frame_MIR:5 ↔ m4 nuts_MIR:28
- Insert:248: servo handle 4_MIR:5 ↔ m2x8_MIR:17
- Insert:249: servo handle 4_MIR:5 ↔ m2x8_MIR:18
- Insert:250: servo handle 4_MIR:5 ↔ m2x8_MIR:19
- Insert:251: servo handle 4_MIR:5 ↔ m2x8_MIR:20
- Mate:134: servo frame mg996r_MIR:3 ↔ servo frame part 3_MIR:2
- Mate:135: servo frame mg996r_MIR:3 ↔ servo frame part 3_MIR:2
- Mate:136: servo frame mg996r_MIR:3 ↔ servo frame part 3_MIR:2
- Mate:137: servo frame mg996r_MIR:3 ↔ servo frame part 3_MIR:2
- Mate:138: servo frame_MIR:5 ↔ servo frame part 3_MIR:2
- Mate:139: servo frame_MIR:5 ↔ servo frame part 3_MIR:2
- Mate:140: servo frame_MIR:5 ↔ servo frame part 3_MIR:2
- Mate:141: servo handle 4_MIR:5 ↔ servo frame mg996 foot_MIR_MIR:1
- Mate:142: m2x8_MIR:18 ↔ servo frame mg996 foot_MIR_MIR:1
- Mate:143: m2x8_MIR:19 ↔ servo frame mg996 foot_MIR_MIR:1
- Rotational:1 [RevoluteJoint]: servo-motor-mg996r servo:1 ↔ servo handle 4:1
- [RevoluteJoint]: servo-motor-mg996r servo:2 ↔ servo handle 4:2
- [RevoluteJoint]: servo-motor-mg996r servo:3 ↔ servo handle 4:3
- [RevoluteJoint]: servo-motor-mg996r servo:4 ↔ servo handle 4:4
- [RevoluteJoint]: servo-motor-mg996r servo:5 ↔ servo handle 4:5
- [RevoluteJoint]: servo-motor-mg996r servo:6 ↔ servo handle 4:6
- [RevoluteJoint]: servo-motor-mg996r servo:10 ↔ servo handle 4:10
- Rotational:11 [RevoluteJoint]: servo-motor-mg996r servo_MIR:1 ↔ servo handle 4_MIR:1
- Rotational:12 [RevoluteJoint]: servo-motor-mg996r servo_MIR:2 ↔ servo handle 4_MIR:2
- Rotational:13 [RevoluteJoint]: servo-motor-mg996r servo_MIR:3 ↔ servo handle 4_MIR:3
- Rotational:14 [RevoluteJoint]: servo-motor-mg996r servo_MIR:4 ↔ servo handle 4_MIR:4
- Rotational:15 [RevoluteJoint]: servo-motor-mg996r servo_MIR:5 ↔ servo handle 4_MIR:5
- Mate:144: servo handle 4:10 ↔ servo frame mg996 centered_MIR_MIR:1
- Mate:146: servo frame mg996 centered_MIR:1 ↔ m2x8:23
- Insert:252: servo handle 4:10 ↔ m2x8:41
- Insert:253: servo handle 4:10 ↔ m2x8:43
- Insert:254: servo handle 4:10 ↔ m2x8:44
- Insert:255: servo handle 4:10 ↔ m2x8:42
- Mate:147: servo frame mg996 centered_MIR_MIR:1 ↔ m2x8:43
- Mate:148: servo frame mg996 centered_MIR_MIR:1 ↔ m2x8:42
- Insert:256: servo frame part 4:1 ↔ m3x8:20
- Insert:257: servo frame part 4:1 ↔ m3x8:19
- Insert:258: servo frame part 4:1 ↔ m3x8:18
- Insert:259: servo frame part 4:1 ↔ m3x8:16
- Insert:260: servo frame part 4:1 ↔ m3x8:17
- Insert:261: servo frame part 4:2 ↔ m3x8:40
- Insert:262: servo frame part 4:2 ↔ m3x8:39
- Insert:263: servo frame part 4:2 ↔ m3x8:36
- Insert:264: servo frame part 4:2 ↔ m3x8:4
- Insert:265: servo frame part 4:2 ↔ m3x8:3
- Insert:266: servo frame part 4:2 ↔ m3x8:5
- Insert:267: servo frame part 4:2 ↔ m3x8:38
- Insert:268: servo frame part 4:2 ↔ m3x8:37
- Insert:269: servo frame part 4:2 ↔ m3x8:1
- Insert:270: servo frame part 4:2 ↔ m3x8:2
- Insert:271: servo frame part 4:1 ↔ m3x8:11
- Insert:272: servo frame part 4:1 ↔ m3x8:24
- Insert:273: servo frame part 4:1 ↔ m3x8:25
- Insert:274: servo frame part 4:1 ↔ m3x8:9
- Insert:275: servo frame part 4:1 ↔ m3x8:10
- Insert:276: servo frame mg996r_MIR:1 ↔ m3x8:6
- Insert:277: servo frame mg996r_MIR:1 ↔ m3x8:7
- Insert:278: servo frame mg996r_MIR:1 ↔ m3x8:8
- Insert:279: servo frame mg996r_MIR:1 ↔ m3x8:23
- Insert:280: servo frame mg996r_MIR:1 ↔ m3x8:21
- Insert:281: servo frame mg996r:1 ↔ m3x8:15
- Insert:282: servo frame mg996r:1 ↔ m3x8:14
- Insert:283: servo frame mg996r:1 ↔ m3x8:13
- Insert:284: servo frame mg996r:1 ↔ m3x8:12
- Insert:285: servo frame mg996r:1 ↔ m3x8:22
- Insert:286: servo frame part 3:1 ↔ m3x8:30
- Insert:287: servo frame part 3:1 ↔ m3x8:29
- Insert:288: servo frame part 3:1 ↔ m3x8:28
- Insert:289: servo frame part 3:1 ↔ m3x8:27
- Insert:290: servo frame part 3:1 ↔ m3x8:26
- Insert:291: servo frame:2 ↔ m3x8:66
- Insert:292: servo frame:2 ↔ m3x8:67
- Insert:293: servo frame:2 ↔ m3x8:68
- Insert:294: servo frame:2 ↔ m3x8:69
- Insert:295: servo frame:2 ↔ m3x8:70
- Insert:296: servo frame mg996r:3 ↔ m3x8:51
- Insert:297: servo frame mg996r:3 ↔ m3x8:52
- Insert:298: servo frame mg996r:3 ↔ m3x8:41
- Insert:299: servo frame mg996r:3 ↔ m3x8:43
- Insert:300: servo frame mg996r:3 ↔ m3x8:42
- Insert:301: servo frame mg996r_MIR:3 ↔ m3x8:44
- Insert:302: servo frame mg996r_MIR:3 ↔ m3x8:65
- Insert:303: servo frame mg996r_MIR:3 ↔ m3x8:61
- Insert:304: servo frame mg996r_MIR:3 ↔ m3x8:64
- Insert:305: servo frame mg996r_MIR:3 ↔ m3x8:45
- Insert:306: servo frame_MIR:2 ↔ m3x8:31
- Insert:307: servo frame_MIR:2 ↔ m3x8:46
- Insert:308: servo frame_MIR:2 ↔ m3x8:53
- Insert:309: servo frame_MIR:2 ↔ m3x8:54
- Insert:310: servo frame_MIR:2 ↔ m3x8:55
- Insert:311: servo frame part 3_MIR:1 ↔ m3x8:34
- Insert:312: servo frame part 3_MIR:1 ↔ m3x8:47
- Insert:313: servo frame part 3_MIR:1 ↔ m3x8:48
- Insert:314: servo frame part 3_MIR:1 ↔ m3x8:50
- Insert:315: servo frame part 3_MIR:1 ↔ m3x8:49
- Insert:316: servo frame part 3:1 ↔ m3x8:80
- Insert:317: servo frame part 3:1 ↔ m3x8:79
- Insert:318: servo frame part 3:1 ↔ m3x8:74
- Insert:319: servo frame part 3:1 ↔ m3x8:78
- Insert:320: servo frame part 3:1 ↔ m3x8:77
- Insert:321: servo frame part 3:1 ↔ m3x8:71
- Insert:322: servo frame part 3:1 ↔ m3x8:75
- Insert:323: servo frame part 3:1 ↔ m3x8:72
- Insert:324: servo frame part 3:1 ↔ m3x8:76
- Insert:325: servo frame part 3:1 ↔ m3x8:73
- Insert:326: servo frame part 3_MIR:1 ↔ m3x8:60
- Insert:327: servo frame part 3_MIR:1 ↔ m3x8:59
- Insert:328: servo frame part 3_MIR:1 ↔ m3x8:58
- Insert:329: servo frame part 3_MIR:1 ↔ m3x8:33
- Insert:330: servo frame part 3_MIR:1 ↔ m3x8:32
- Insert:331: servo frame part 3_MIR:1 ↔ m3x8:98
- Insert:332: servo frame part 3_MIR:1 ↔ m3x8:99
- Insert:333: servo frame part 3_MIR:1 ↔ m3x8:100
- Insert:334: servo frame part 3_MIR:1 ↔ m3x8:97
- Insert:335: servo frame part 3_MIR:1 ↔ m3x8:96
- Insert:336: servo frame part 3_MIR:2 ↔ m3x8:62
- Insert:337: servo frame part 3_MIR:2 ↔ m3x8:63
- Insert:338: servo frame part 3_MIR:2 ↔ m3x8:84
- Insert:339: servo frame part 3_MIR:2 ↔ m3x8:85
- Insert:340: servo frame part 3_MIR:2 ↔ m3x8:56
- Insert:341: servo frame part 3_MIR:2 ↔ m3x8:57
- Insert:342: servo frame part 3_MIR:2 ↔ m3x8:35
- Insert:343: servo frame part 3_MIR:2 ↔ m3x8:82
- Insert:344: servo frame part 3_MIR:2 ↔ m3x8:81
- Insert:345: servo frame part 3_MIR:2 ↔ m3x8:83
- Insert:346: servo frame part 3:2 ↔ m3x8:95
- Insert:347: servo frame part 3:2 ↔ m3x8:89
- Insert:348: servo frame part 3:2 ↔ m3x8:90
- Insert:349: servo frame part 3:2 ↔ m3x8:94
- Insert:350: servo frame part 3:2 ↔ m3x8:87
- Insert:351: servo frame part 3:2 ↔ m3x8:93
- Insert:352: servo frame part 3:2 ↔ m3x8:91
- Insert:353: servo frame part 3:2 ↔ m3x8:86
- Insert:354: servo frame part 3:2 ↔ m3x8:88
- Insert:355: servo frame part 3:2 ↔ m3x8:92
- Insert:356: servo frame:6 ↔ m3 nuts:6
- Insert:357: servo frame:6 ↔ m3 nuts:7
- Insert:358: servo frame:6 ↔ m3 nuts:1
- Insert:359: servo frame:6 ↔ m3 nuts:2
- Insert:360: servo frame:6 ↔ m3 nuts:8
- Insert:361: servo frame:6 ↔ m3 nuts:4
- Insert:362: servo frame:6 ↔ m3 nuts:5
- Insert:363: servo frame:6 ↔ m3 nuts:9
- Insert:364: servo frame:6 ↔ m3 nuts:10
- Insert:365: servo frame:6 ↔ m3 nuts:3
- Insert:366: servo frame:10 ↔ m3 nuts:35
- Insert:367: servo frame:10 ↔ m3 nuts:23
- Insert:368: servo frame:10 ↔ m3 nuts:39
- Insert:369: servo frame:10 ↔ m3 nuts:17
- Insert:370: servo frame:10 ↔ m3 nuts:34
- Insert:371: servo frame:10 ↔ m3 nuts:24
- Insert:372: servo frame:10 ↔ m3 nuts:33
- Insert:373: servo frame:10 ↔ m3 nuts:40
- Insert:374: servo frame:10 ↔ m3 nuts:90
- Insert:375: servo frame:10 ↔ m3 nuts:41
- Insert:376: servo frame:1 ↔ m3 nuts:29
- Insert:377: servo frame:1 ↔ m3 nuts:51
- Insert:378: servo frame:1 ↔ m3 nuts:46
- Insert:379: servo frame:1 ↔ m3 nuts:18
- Insert:380: servo frame:1 ↔ m3 nuts:30
- Insert:381: servo frame_MIR:1 ↔ m3 nuts:22
- Insert:382: servo frame_MIR:1 ↔ m3 nuts:53
- Insert:383: servo frame_MIR:1 ↔ m3 nuts:52
- Insert:384: servo frame_MIR:1 ↔ m3 nuts:47
- Insert:385: servo frame_MIR:1 ↔ m3 nuts:13
- Insert:386: servo frame mg996r:2 ↔ m3 nuts:28
- Insert:387: servo frame mg996r:2 ↔ m3 nuts:38
- Insert:388: servo frame mg996r:2 ↔ m3 nuts:45
- Insert:389: servo frame mg996r:2 ↔ m3 nuts:11
- Insert:390: servo frame mg996r:2 ↔ m3 nuts:19
- Insert:391: servo frame mg996r_MIR:2 ↔ m3 nuts:25
- Insert:392: servo frame mg996r_MIR:2 ↔ m3 nuts:16
- Insert:393: servo frame mg996r_MIR:2 ↔ m3 nuts:44
- Insert:394: servo frame mg996r_MIR:2 ↔ m3 nuts:12
- Insert:395: servo frame mg996r_MIR:2 ↔ m3 nuts:42
- Insert:396: servo frame:3 ↔ m3 nuts:43
- Insert:397: servo frame:3 ↔ m3 nuts:26
- Insert:398: servo frame:3 ↔ m3 nuts:21
- Insert:399: servo frame:3 ↔ m3 nuts:31
- Insert:400: servo frame:3 ↔ m3 nuts:36
- Insert:401: servo frame_MIR:3 ↔ m3 nuts:14
- Insert:402: servo frame_MIR:3 ↔ m3 nuts:27
- Insert:403: servo frame_MIR:3 ↔ m3 nuts:37
- Insert:404: servo frame_MIR:3 ↔ m3 nuts:32
- Insert:405: servo frame_MIR:3 ↔ m3 nuts:79
- Insert:406: servo frame:4 ↔ m3 nuts:73
- Insert:407: servo frame:4 ↔ m3 nuts:83
- Insert:408: servo frame:4 ↔ m3 nuts:84
- Insert:409: servo frame:4 ↔ m3 nuts:80
- Insert:410: servo frame:4 ↔ m3 nuts:78
- Insert:411: servo frame:4 ↔ m3 nuts:74
- Insert:412: servo frame:4 ↔ m3 nuts:85
- Insert:413: servo frame:4 ↔ m3 nuts:86
- Insert:414: servo frame:4 ↔ m3 nuts:68
- Insert:415: servo frame:4 ↔ m3 nuts:49
- Insert:416: servo frame_MIR:4 ↔ m3 nuts:67
- Insert:417: servo frame_MIR:4 ↔ m3 nuts:81
- Insert:418: servo frame_MIR:4 ↔ m3 nuts:82
- Insert:419: servo frame_MIR:4 ↔ m3 nuts:77
- Insert:420: servo frame_MIR:4 ↔ m3 nuts:62
- Insert:421: servo frame_MIR:4 ↔ m3 nuts:75
- Insert:422: servo frame_MIR:4 ↔ m3 nuts:63
- Insert:423: servo frame_MIR:4 ↔ m3 nuts:48
- Insert:424: servo frame_MIR:4 ↔ m3 nuts:87
- Insert:425: servo frame_MIR:4 ↔ m3 nuts:61
- Insert:426: servo frame part 3:2 ↔ m3 nuts:56
- Insert:427: servo frame part 3_MIR:2 ↔ m3 nuts:72
- Insert:428: servo frame part 3_MIR:2 ↔ m3 nuts:89
- Insert:429: servo frame part 3_MIR:2 ↔ m3 nuts:76
- Insert:430: servo frame part 3:2 ↔ m3 nuts:66
- Insert:431: servo frame part 3:2 ↔ m3 nuts:60
- Insert:432: servo frame part 3:2 ↔ m3 nuts:57
- Insert:433: servo frame part 3:2 ↔ m3 nuts:20
- Insert:434: servo frame part 3_MIR:2 ↔ m3 nuts:88
- Insert:435: servo frame part 3_MIR:2 ↔ m3 nuts:69
- Insert:436: servo frame:5 ↔ m3 nuts:71
- Insert:437: servo frame:5 ↔ m3 nuts:70
- Insert:438: servo frame:5 ↔ m3 nuts:50
- Insert:439: servo frame:5 ↔ m3 nuts:54
- Insert:440: servo frame:5 ↔ m3 nuts:15
- Insert:441: servo frame_MIR:5 ↔ m3 nuts:95
- Insert:442: servo frame_MIR:5 ↔ m3 nuts:93
- Insert:443: servo frame_MIR:5 ↔ m3 nuts:94
- Insert:444: servo frame_MIR:5 ↔ m3 nuts:92
- Insert:445: servo frame_MIR:5 ↔ m3 nuts:91
- Insert:446: servo frame:5 ↔ m3 nuts:99
- Insert:447: servo frame:5 ↔ m3 nuts:96
- Insert:448: servo frame:5 ↔ m3 nuts:98
- Insert:449: servo frame:5 ↔ m3 nuts:97
- Insert:450: servo frame:5 ↔ m3 nuts:100
- Insert:451: servo frame_MIR:5 ↔ m3 nuts:64
- Insert:452: servo frame_MIR:5 ↔ m3 nuts:58
- Insert:453: servo frame_MIR:5 ↔ m3 nuts:65
- Insert:454: servo frame_MIR:5 ↔ m3 nuts:55
- Insert:455: servo frame_MIR:5 ↔ m3 nuts:59
- Insert:456: servo frame mg996 centered_MIR:1 ↔ m4 nuts:56
- Insert:457: servo frame mg996 centered_MIR_MIR:1 ↔ m4 nuts:57
- Insert:458: servo frame mg996 foot_MIR:1 ↔ m4 nuts:55
- Insert:459: servo frame mg996 foot_MIR_MIR:1 ↔ m4 nuts:58
- Insert:460: servo frame mg996 foot_MIR:1 ↔ m2 nuts:20
- Insert:461: servo frame mg996 foot_MIR:1 ↔ m2 nuts:19
- Insert:462: servo frame mg996 foot_MIR:1 ↔ m2 nuts:16
- Insert:463: servo frame mg996 foot_MIR:1 ↔ m2 nuts:15
- Insert:464: servo frame mg996 foot_MIR_MIR:1 ↔ m2 nuts:13
- Insert:465: servo frame mg996 foot_MIR_MIR:1 ↔ m2 nuts:14
- Insert:466: servo frame mg996 foot_MIR_MIR:1 ↔ m2 nuts:33
- Insert:467: servo frame mg996 foot_MIR_MIR:1 ↔ m2 nuts:36
- Insert:468: servo frame mg996 centered_MIR:1 ↔ m2 nuts:21
- Insert:469: servo frame mg996 centered_MIR:1 ↔ m2 nuts:32
- Insert:470: servo frame mg996 centered_MIR:1 ↔ m2 nuts:18
- Insert:471: servo frame mg996 centered_MIR:1 ↔ m2 nuts:25
- Insert:472: servo frame mg996 centered_MIR_MIR:1 ↔ m2 nuts:27
- Insert:473: servo frame mg996 centered_MIR_MIR:1 ↔ m2 nuts:34
- Insert:474: servo frame mg996 centered_MIR_MIR:1 ↔ m2 nuts:35
- Insert:475: servo frame mg996 centered_MIR_MIR:1 ↔ m2 nuts:26
- Insert:476: servo frame mg996 centered_MIR:1 ↔ m2 nuts:31
- Insert:477: servo frame mg996 centered_MIR:1 ↔ m2 nuts:17
- Insert:478: servo frame mg996 centered_MIR:1 ↔ m2 nuts:30
- Insert:479: servo frame mg996 centered_MIR:1 ↔ m2 nuts:29
- Insert:480: servo frame mg996 centered_MIR_MIR:1 ↔ m2 nuts:22
- Insert:481: servo frame mg996 centered_MIR_MIR:1 ↔ m2 nuts:24
- Insert:482: servo frame mg996 centered_MIR_MIR:1 ↔ m2 nuts:28